# Autodesk Inventor assembly: LR2_Assemblie
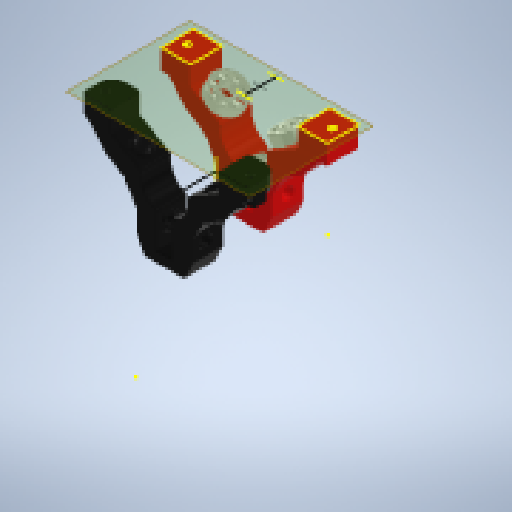
[picture p0: Inventor's stored thumbnail of the model, 512x512]
Saved by Autodesk Inventor 2024 (Build 280153000, 153)
## iProperties
Created: 2023-11-24
Part Number: LR2_Assemblie
Document SubType Name: Assembly
Designer: danie
Author: danie
## Documents named in this file (4)
- C:\GitHubDesktop\3d-model\basis_roboter\low_rider_v2\custom_files\LR2_Assemblie.iam
- C:\GitHubDesktop\3d-model\Imported Components\LR2_X_mount\LR2_X_mount.ipt
- C:\GitHubDesktop\3d-model\basis_roboter\low_rider_v2\custom_files\Bearing.ipt
- C:\Users\danie\OneDrive\Documents\Inventor\Content Center Files\R2023\en-US\ISO 8674(2)\ISO 8674 - M8 x 1ISO.ipt
## Components (6 placed, 3 different names)
1. LR2_X_mount:1 — Rigid:1, Mate:4, Rigid:2, Mate:7, Mate:8, Rigid:3
2. Bearing:1 — Rigid:1, Mate:3
3. ISO 8674 M8 x 1:1 — Mate:3, Mate:4
4. Bearing:2 — Rigid:2
5. ISO 8674 M8 x 1:2 — Mate:7, Mate:8
6. Bearing:3 — Rigid:3
## Relationships (7: Mate 4, WeldJoint 3)
- Rigid:1 [WeldJoint]: LR2_X_mount:1 ↔ Bearing:1
- Mate:3: Bearing:1 ↔ ISO 8674 M8 x 1:1
- Mate:4: LR2_X_mount:1 ↔ ISO 8674 M8 x 1:1
- Rigid:2 [WeldJoint]: LR2_X_mount:1 ↔ Bearing:2
- Mate:7: LR2_X_mount:1 ↔ ISO 8674 M8 x 1:2
- Mate:8: LR2_X_mount:1 ↔ ISO 8674 M8 x 1:2
- Rigid:3 [WeldJoint]: LR2_X_mount:1 ↔ Bearing:3
